# Autodesk Inventor assembly: Foot
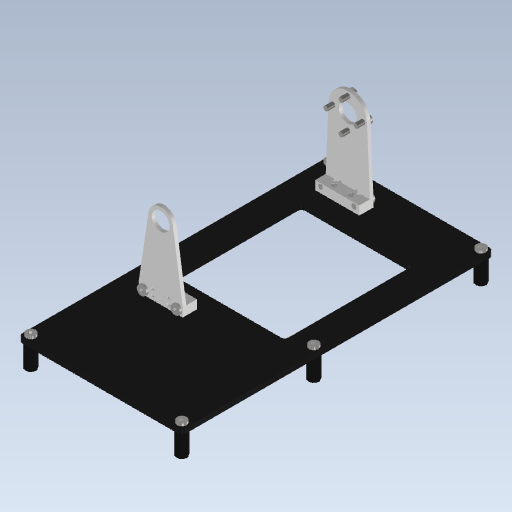
[picture p0: Inventor's stored thumbnail of the model, 512x512]
Saved by Autodesk Inventor 2020.4 (Build 244396000, 396)
## iProperties
Created: 2022-01-10
Part Number: Foot
Document SubType Name: Assembly
Designer: Masato Kubotera
Author: Masato Kubotera
## Documents named in this file (9)
- C:\Users\Masato\Documents\Inventor\CIT Brains_Inventor\OpenPlatform_ver3_0\LowerBody\Foot\Foot.iam
- C:\Users\Masato\Documents\Inventor\CIT Brains_Inventor\OpenPlatform_ver3_0\LowerBody\Foot\Foot_back_frame.ipt
- C:\Users\Masato\Documents\Inventor\CIT Brains_Inventor\OpenPlatform_ver3_0\LowerBody\Foot\Foot_front_frame.ipt
- C:\Users\Masato\Documents\Inventor\CIT Brains_Inventor\OpenPlatform_ver3_0\LowerBody\Foot\Foot_root_block.ipt
- C:\Users\Masato\Documents\Inventor\CIT Brains_Inventor\OpenPlatform_ver3_0\LowerBody\Foot\Sole_frame.ipt
- C:\Users\Masato\Documents\Inventor\CIT Brains_Inventor\OpenPlatform_ver3_0\ReadyMade\Spacer\ASL-313BE.ipt
- C:\Users\Masato\Documents\Inventor\CIT Brains_Inventor\OpenPlatform_ver3_0\ReadyMade\Screw\M2_6-6.ipt
- C:\Users\Masato\Documents\Inventor\CIT Brains_Inventor\OpenPlatform_ver3_0\ReadyMade\Screw\M3-8.ipt
- C:\Users\Masato\Documents\Inventor\CIT Brains_Inventor\OpenPlatform_ver3_0\ReadyMade\Screw\M3-10.ipt
## Components (29 placed, 8 different names)
1. Sole_frame:1 — フラッシュ:1, フラッシュ:2, フラッシュ:3, 挿入:1, 挿入:2, 挿入:3, 挿入:4, 挿入:9, 挿入:10, 挿入:11, 挿入:12, 挿入:13, 挿入:14, 角度:1, 挿入:23, 挿入:24, 挿入:25, 挿入:26, 挿入:27, 挿入:28, 挿入:29, 挿入:30, 挿入:31, 挿入:32
2. Foot_back_frame:1 — 挿入:5, 挿入:6, 挿入:15, 挿入:16, 挿入:17, 挿入:18, 挿入:19, 挿入:20
3. Foot_front_frame:1 — 挿入:7, 挿入:8, 挿入:21, 挿入:22
4. Foot_root_block:1 — 挿入:1, 挿入:2, 挿入:5, 挿入:6
5. Foot_root_block:2 — 挿入:3, 挿入:4, 挿入:7, 挿入:8
6. ASL-313BE:1 — 挿入:9, 角度:1, 角度:2, 角度:3, 角度:4, 角度:5, 角度:6
7. ASL-313BE:2 — 挿入:10, 角度:2
8. ASL-313BE:3 — 挿入:11, 角度:3
9. ASL-313BE:4 — 挿入:12, 角度:4
10. ASL-313BE:5 — 挿入:13, 角度:5
11. ASL-313BE:6 — 挿入:14, 角度:6
12. M2_6-6:1 — 挿入:15
13. M2_6-6:2 — 挿入:16
14. M2_6-6:3 — 挿入:17
15. M2_6-6:4 — 挿入:18
16. M3-8:1 — 挿入:19
17. M3-8:2 — 挿入:20
18. M3-8:3 — 挿入:21
19. M3-8:4 — 挿入:22
20. M3-8:5 — 挿入:23
21. M3-8:6 — 挿入:24
22. M3-8:7 — 挿入:25
23. M3-8:8 — 挿入:26
24. M3-10:1 — 挿入:27
25. M3-10:2 — 挿入:28
26. M3-10:3 — 挿入:29
27. M3-10:4 — 挿入:30
28. M3-10:5 — 挿入:31
29. M3-10:6 — 挿入:32
## Relationships (41: Insert 32, Angle 6, Flush 3)
- フラッシュ:1 [Flush]: Sole_frame:1
- フラッシュ:2 [Flush]: Sole_frame:1
- フラッシュ:3 [Flush]: Sole_frame:1
- 挿入:1 [Insert]: Sole_frame:1 ↔ Foot_root_block:1
- 挿入:2 [Insert]: Sole_frame:1 ↔ Foot_root_block:1
- 挿入:3 [Insert]: Sole_frame:1 ↔ Foot_root_block:2
- 挿入:4 [Insert]: Sole_frame:1 ↔ Foot_root_block:2
- 挿入:5 [Insert]: Foot_back_frame:1 ↔ Foot_root_block:1
- 挿入:6 [Insert]: Foot_back_frame:1 ↔ Foot_root_block:1
- 挿入:7 [Insert]: Foot_front_frame:1 ↔ Foot_root_block:2
- 挿入:8 [Insert]: Foot_front_frame:1 ↔ Foot_root_block:2
- 挿入:9 [Insert]: Sole_frame:1 ↔ ASL-313BE:1
- 挿入:10 [Insert]: Sole_frame:1 ↔ ASL-313BE:2
- 挿入:11 [Insert]: Sole_frame:1 ↔ ASL-313BE:3
- 挿入:12 [Insert]: Sole_frame:1 ↔ ASL-313BE:4
- 挿入:13 [Insert]: Sole_frame:1 ↔ ASL-313BE:5
- 挿入:14 [Insert]: Sole_frame:1 ↔ ASL-313BE:6
- 角度:1 [Angle] (0 deg): Sole_frame:1 ↔ ASL-313BE:1
- 角度:2 [Angle] (0 deg): ASL-313BE:1 ↔ ASL-313BE:2
- 角度:3 [Angle] (0 deg): ASL-313BE:1 ↔ ASL-313BE:3
- 角度:4 [Angle] (0 deg): ASL-313BE:1 ↔ ASL-313BE:4
- 角度:5 [Angle] (0 deg): ASL-313BE:1 ↔ ASL-313BE:5
- 角度:6 [Angle] (0 deg): ASL-313BE:1 ↔ ASL-313BE:6
- 挿入:15 [Insert]: Foot_back_frame:1 ↔ M2_6-6:1
- 挿入:16 [Insert]: Foot_back_frame:1 ↔ M2_6-6:2
- 挿入:17 [Insert]: Foot_back_frame:1 ↔ M2_6-6:3
- 挿入:18 [Insert]: Foot_back_frame:1 ↔ M2_6-6:4
- 挿入:19 [Insert]: Foot_back_frame:1 ↔ M3-8:1
- 挿入:20 [Insert]: Foot_back_frame:1 ↔ M3-8:2
- 挿入:21 [Insert]: Foot_front_frame:1 ↔ M3-8:3
- 挿入:22 [Insert]: Foot_front_frame:1 ↔ M3-8:4
- 挿入:23 [Insert]: Sole_frame:1 ↔ M3-8:5
- 挿入:24 [Insert]: Sole_frame:1 ↔ M3-8:6
- 挿入:25 [Insert]: Sole_frame:1 ↔ M3-8:7
- 挿入:26 [Insert]: Sole_frame:1 ↔ M3-8:8
- 挿入:27 [Insert]: Sole_frame:1 ↔ M3-10:1
- 挿入:28 [Insert]: Sole_frame:1 ↔ M3-10:2
- 挿入:29 [Insert]: Sole_frame:1 ↔ M3-10:3
- 挿入:30 [Insert]: Sole_frame:1 ↔ M3-10:4
- 挿入:31 [Insert]: Sole_frame:1 ↔ M3-10:5
- 挿入:32 [Insert]: Sole_frame:1 ↔ M3-10:6
